# Autodesk Inventor assembly: Truc
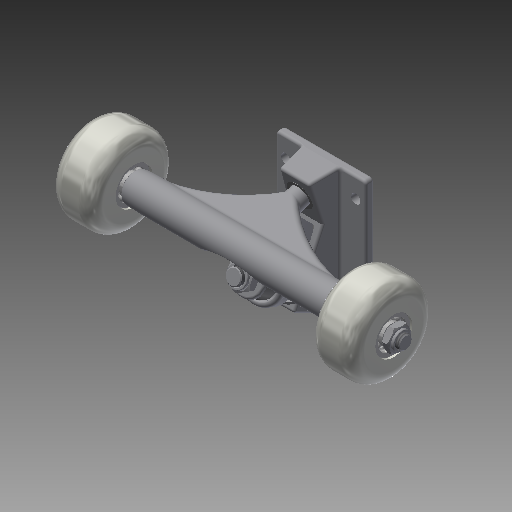
[picture p0: Inventor's stored thumbnail of the model, 512x512]
Saved by Autodesk Inventor 2019 (Build 230136000, 136)
## iProperties
Created: 2011-10-06
Part Number: Truc
Document SubType Name: Assembly
Designer: Stefano
Author: Stefano
## Documents named in this file (13)
- C:\Users\drago\Documents\SFP\sfp_smartboard\track_data\Truck.iam
- C:\Users\drago\Documents\SFP\sfp_smartboard\track_data\Basetta.ipt
- C:\Users\drago\Documents\SFP\sfp_smartboard\track_data\Dado 14.ipt
- C:\Users\drago\Documents\SFP\sfp_smartboard\track_data\Gommino inferiore.ipt
- C:\Users\drago\Documents\SFP\sfp_smartboard\track_data\Gommino superiore.ipt
- C:\Users\drago\Documents\SFP\sfp_smartboard\track_data\Kingpin.ipt
- C:\Users\drago\Documents\SFP\sfp_smartboard\track_data\Rondella inferiore.ipt
- C:\Users\drago\Documents\SFP\sfp_smartboard\track_data\Rondella superiore.ipt
- C:\Users\drago\Documents\SFP\sfp_smartboard\track_data\Hanger.ipt
- C:\Users\drago\Documents\SFP\sfp_smartboard\track_data\Rondella.ipt
- C:\Users\drago\Documents\SFP\sfp_smartboard\track_data\Ruota.ipt
- C:\Users\drago\Documents\SFP\sfp_smartboard\track_data\Dado 13.ipt
- C:\Users\drago\Documents\SFP\sfp_smartboard\track_data\Cuscinetto CC.ipt
## Components (20 placed, 12 different names)
1. Basetta:1 — Perno/foro:1, Perno/foro:5, Coincidente:3
2. Dado 14:1 — Coincidente:1, Coincidente:2
3. Gommino inferiore:1 — Perno/foro:6, Perno/foro:7
4. Gommino superiore:1 — Perno/foro:3
5. Kingpin:1 — Perno/foro:1, Coincidente:1
6. Rondella inferiore:1 — Perno/foro:5, Perno/foro:6
7. Rondella superiore:1 — Perno/foro:3, Coincidente:2
8. Hanger2:1 — Perno/foro:7, Coincidente:3, Perno/foro:8, Perno/foro:9, Coincidente:11, Coincidente:25, Coincidente:32
9. Rondella:1 — Perno/foro:9, Perno/foro:16
10. Rondella:2 — Coincidente:25, Coincidente:27, Perno/foro:17
11. Rondella:3 — Coincidente:30, Coincidente:33, Perno/foro:13
12. Rondella:4 — Perno/foro:8, Perno/foro:10
13. Ruota:1 — Perno/foro:14, Perno/foro:15
14. Ruota:2 — Coincidente:32, Perno/foro:11, Perno/foro:12
15. Dado 13:1 — Coincidente:11, Coincidente:27
16. Dado 13:2 — Coincidente:30, Coincidente:33
17. DIN 625 SKF- con schermatura Z SKF 608-Z:1 — Perno/foro:10, Perno/foro:11
18. DIN 625 SKF- con schermatura Z SKF 608-Z:2 — Perno/foro:15, Perno/foro:16
19. DIN 625 SKF- con schermatura Z SKF 608-Z:3 — Perno/foro:12, Perno/foro:13
20. DIN 625 SKF- con schermatura Z SKF 608-Z:4 — Perno/foro:14, Perno/foro:17
## Relationships (24: Insert 15, Mate 9)
- Perno/foro:1 [Insert]: Basetta:1 ↔ Kingpin:1
- Perno/foro:3 [Insert]: Gommino superiore:1 ↔ Rondella superiore:1
- Perno/foro:5 [Insert]: Basetta:1 ↔ Rondella inferiore:1
- Perno/foro:6 [Insert]: Gommino inferiore:1 ↔ Rondella inferiore:1
- Coincidente:1 [Mate]: Dado 14:1 ↔ Kingpin:1
- Coincidente:2 [Mate]: Dado 14:1 ↔ Rondella superiore:1
- Perno/foro:7 [Insert]: Gommino inferiore:1 ↔ Hanger2:1
- Coincidente:3 [Mate]: Basetta:1 ↔ Hanger2:1
- Perno/foro:8 [Insert]: Hanger2:1 ↔ Rondella:4
- Perno/foro:9 [Insert]: Hanger2:1 ↔ Rondella:1
- Coincidente:11 [Mate]: Hanger2:1 ↔ Dado 13:1
- Coincidente:25 [Mate]: Hanger2:1 ↔ Rondella:2
- Coincidente:27 [Mate]: Rondella:2 ↔ Dado 13:1
- Coincidente:30 [Mate]: Rondella:3 ↔ Dado 13:2
- Coincidente:32 [Mate]: Hanger2:1 ↔ Ruota:2
- Coincidente:33 [Mate]: Rondella:3 ↔ Dado 13:2
- Perno/foro:10 [Insert]: Rondella:4 ↔ DIN 625 SKF- con schermatura Z SKF 608-Z:1
- Perno/foro:11 [Insert]: Ruota:2 ↔ DIN 625 SKF- con schermatura Z SKF 608-Z:1
- Perno/foro:12 [Insert]: Ruota:2 ↔ DIN 625 SKF- con schermatura Z SKF 608-Z:3
- Perno/foro:13 [Insert]: Rondella:3 ↔ DIN 625 SKF- con schermatura Z SKF 608-Z:3
- Perno/foro:14 [Insert]: Ruota:1 ↔ DIN 625 SKF- con schermatura Z SKF 608-Z:4
- Perno/foro:15 [Insert]: Ruota:1 ↔ DIN 625 SKF- con schermatura Z SKF 608-Z:2
- Perno/foro:16 [Insert]: Rondella:1 ↔ DIN 625 SKF- con schermatura Z SKF 608-Z:2
- Perno/foro:17 [Insert]: Rondella:2 ↔ DIN 625 SKF- con schermatura Z SKF 608-Z:4
